# Autodesk Inventor assembly: A1-19027-200-00 Spool
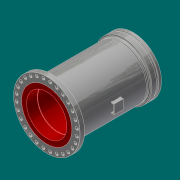
[picture p0: Inventor's stored thumbnail of the model, 180x180]
Saved by Autodesk Inventor 2017.3 (Build 213257000, 257)
## iProperties
Created: 2019-06-26
Part Number: A1-19027-200-00 Spool
Document SubType Name: Weldment
Designer: Graeme_Van_Dongen
Mass: 1.99002e+06 g
Surface Area: 164280 cm^2
Volume: 265271 cm^3
Density: 7.50182 g/cm^3
Weld Material: Steel, Mild, Welded
Author: Graeme_Van_Dongen
## Documents named in this file (6)
- N:\A1 - Projects\A1-19\A1-19027--Syncrude Aurora HT2 spools - SP-237\A1-19027-200-00 Spool SP-237-002-P-002-1-A.iam
- N:\A1 - Projects\A1-19\A1-19027--Syncrude Aurora HT2 spools - SP-237\A1-19027-200-03 30in CL250 flange.ipt
- N:\A1 - Projects\A1-19\A1-19027--Syncrude Aurora HT2 spools - SP-237\A1-19027-200-04 HCWi reducer.ipt
- N:\A1 - Projects\A1-19\A1-19027--Syncrude Aurora HT2 spools - SP-237\A1-19027-200-01 34in pipe.ipt
- N:\A1 - Projects\A1-19\A1-19027--Syncrude Aurora HT2 spools - SP-237\A1-19027-200-02 34in Type B victaulic ring.ipt
- N:\Penticton Foundry\Tag mount - 6in.ipt
## Components (6 placed, 5 different names)
1. A1-19027-200-01 34in pipe:1 — Insert:1, Angle:1, Angle:3, Insert:5, Angle:4, Flush:1, Tangent:1
2. A1-19027-200-02 34in Type B victaulic ring:1 — Insert:1, Angle:1, Insert:4, Flush:2
3. A1-19027-200-03 30in CL250 flange:1 — Angle:3, Insert:5
4. A1-19027-200-04 HCWi reducer:1 — Insert:4, Angle:4
5. Tag mount - 6in:1 — Flush:1, Flush:2, Tangent:1
6. Tag mount - 6in:2
## Component patterns: (2 elements, first: Tag mount - 6in:1)
## Relationships (9: Insert 3, Angle 3, Flush 2, Tangent 1)
- Insert:1 (2.3813 mm): A1-19027-200-01 34in pipe:1 ↔ A1-19027-200-02 34in Type B victaulic ring:1
- Angle:1 (0 deg): A1-19027-200-01 34in pipe:1 ↔ A1-19027-200-02 34in Type B victaulic ring:1
- Angle:3 (0 deg): A1-19027-200-01 34in pipe:1 ↔ A1-19027-200-03 30in CL250 flange:1
- Insert:4: A1-19027-200-02 34in Type B victaulic ring:1 ↔ A1-19027-200-04 HCWi reducer:1
- Insert:5 (2.3813 mm): A1-19027-200-01 34in pipe:1 ↔ A1-19027-200-03 30in CL250 flange:1
- Angle:4 (0 deg): A1-19027-200-01 34in pipe:1 ↔ A1-19027-200-04 HCWi reducer:1
- Flush:1: A1-19027-200-01 34in pipe:1 ↔ Tag mount - 6in:1
- Flush:2 (635 mm): A1-19027-200-02 34in Type B victaulic ring:1 ↔ Tag mount - 6in:1
- Tangent:1: A1-19027-200-01 34in pipe:1 ↔ Tag mount - 6in:1
